# Autodesk Inventor assembly: 000 ASY GBK Gubkinskiy
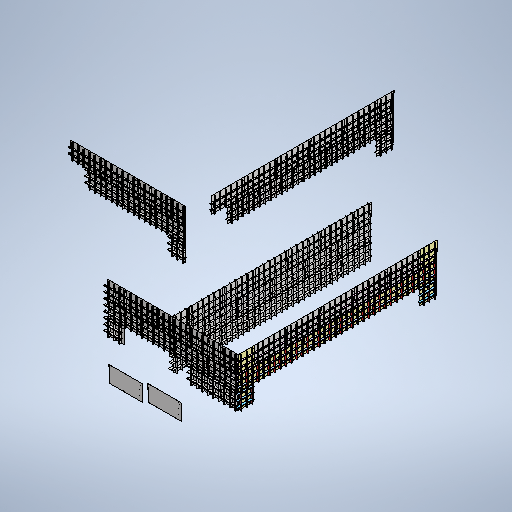
[picture p0: Inventor's stored thumbnail of the model, 512x512]
Saved by Autodesk Inventor 2026.2 (Build 302298010, 298A)
## iProperties
Created: 2026-04-17
Part Number: 000 ASY GBK Gubkinskiy
Document SubType Name: Assembly
Designer: admin
Mass: 2.0116e+07 g
Surface Area: 1.3016e+07 cm^2
Volume: 2.56254e+06 cm^3
Density: 7.85 g/cm^3
Author: admin
## Documents named in this file (20)
- C:\Users\admin\Documents\Inventor\GBK-Gubkinskiy\000 ASY GBK Gubkinskiy.iam
- C:\Users\admin\Documents\Inventor\GBK-Gubkinskiy\GBK bottom.ipt
- C:\Users\admin\Documents\Inventor\GBK-Gubkinskiy\ASY GBK длинная стенка.iam
- C:\Users\admin\Documents\Inventor\GBK-Gubkinskiy\090 ASY bottom.iam
- C:\Users\admin\Documents\Inventor\GBK-Gubkinskiy\ASY GBK короткая стенка.iam
- C:\Users\admin\Documents\Inventor\GBK-Gubkinskiy\ASY GBK центральная стенка.iam
- C:\Users\admin\Documents\Inventor\GBK-Gubkinskiy\ASY GBK 2110 short wall shield 1.iam
- C:\Users\admin\Documents\Inventor\GBK-Gubkinskiy\ASY GBK 2120 short wall shield 2.iam
- C:\Users\admin\Documents\Inventor\GBK-Gubkinskiy\ASY GBK 2130 short wall shield 3.iam
- C:\Users\admin\Documents\Inventor\GBK-Gubkinskiy\ASY GBK 2210 short wall shield 4.iam
- C:\Users\admin\Documents\Inventor\GBK-Gubkinskiy\ASY GBK 2310 short wall shield 7.iam
- C:\Users\admin\Documents\Inventor\GBK-Gubkinskiy\ASY GBK 2320 short wall shield 8.iam
- C:\Users\admin\Documents\Inventor\GBK-Gubkinskiy\ASY GBK 2330 short wall shield 9.iam
- C:\Users\admin\Documents\Inventor\GBK-Gubkinskiy\ASY GBK 2220 short wall shield 5.iam
- C:\Users\admin\Documents\Inventor\GBK-Gubkinskiy\ASY GBK 2230 short wall shield 6.iam
- C:\Users\admin\Documents\Inventor\GBK-Gubkinskiy\ASY GBK 1110 long wall shield 1.iam
- C:\Users\admin\Documents\Inventor\GBK-Gubkinskiy\ASY GBK 1210 long wall shield 3.iam
- C:\Users\admin\Documents\Inventor\GBK-Gubkinskiy\ASY GBK 1310 long wall shield 4.iam
- C:\Users\admin\Documents\Inventor\GBK-Gubkinskiy\ASY GBK 1320 long wall shield 5.iam
- C:\Users\admin\Documents\Inventor\GBK-Gubkinskiy\GBK 2121 shield 2.ipt
## Components (56 placed, 28 different names)
1. GBK bottom.ipt:1 — Flush:8, Flush:9, Mate:20, Mate:21, Flush:14, Mate:23, Flush:19, Flush:21, Flush:22, Mate:24, Mate:25
2. ASY GBK 1110 long wall shield 1.iam:2 [sub-assembly]
3. ASY GBK 1110 long wall shield 1.iam:1 [sub-assembly]
4. ASY GBK 1210 long wall shield 3.iam:1 [sub-assembly]
5. ASY GBK 1310 long wall shield 4.iam:1 [sub-assembly]
6. ASY GBK 1320 long wall shield 5.iam:1 [sub-assembly]
7. ASY GBK 1320 long wall shield 5.iam:2 [sub-assembly]
8. ASY GBK 1320 long wall shield 5.iam:3 [sub-assembly]
9. ASY GBK 1320 long wall shield 5.iam:4 [sub-assembly]
10. ASY GBK 1320 long wall shield 5.iam:5 [sub-assembly]
11. ASY GBK 1210 long wall shield 3.iam:2 [sub-assembly]
12. ASY GBK 1210 long wall shield 3.iam:3 [sub-assembly]
13. ASY GBK 1210 long wall shield 3.iam:4 [sub-assembly]
14. ASY GBK 1210 long wall shield 3.iam:5 [sub-assembly]
15. ASY GBK 1210 long wall shield 3.iam:6 [sub-assembly]
16. ASY GBK 1310 long wall shield 4.iam:2 [sub-assembly]
17. ASY GBK длинная стенка.iam:1 [sub-assembly]
18. ASY GBK длинная стенка.iam:2 [sub-assembly] — Flush:9, Mate:21, Flush:14
19. 090 ASY bottom.iam:1 [sub-assembly] — Mate:19, Flush:8
20. ASY GBK 2110 short wall shield 1.iam:1 [sub-assembly]
21. ASY GBK 2120 short wall shield 2.iam:1 [sub-assembly]
22. ASY GBK 2130 short wall shield 3.iam:1 [sub-assembly]
23. ASY GBK 2210 short wall shield 4.iam:1 [sub-assembly]
24. ASY GBK 2220 short wall shield 5.iam:1 [sub-assembly]
25. ASY GBK 2220 short wall shield 5.iam:2 [sub-assembly]
26. ASY GBK 2230 short wall shield 6.iam:1 [sub-assembly]
27. ASY GBK 2310 short wall shield 7.iam:1 [sub-assembly]
28. ASY GBK 2320 short wall shield 8.iam:1 [sub-assembly]
29. ASY GBK 2330 short wall shield 9.iam:1 [sub-assembly]
30. ASY GBK 2320 short wall shield 8.iam:2 [sub-assembly]
31. ASY GBK 2320 short wall shield 8.iam:3 [sub-assembly]
32. ASY GBK короткая стенка.iam:1 [sub-assembly] — Mate:20, Flush:19, Mate:25, Mate:27
33. ASY GBK короткая стенка.iam:2 [sub-assembly]
34. ASY GBK центральная стенка.iam:1 [sub-assembly] — Mate:23, Flush:18, Mate:27
35. ASY GBK 2110 short wall shield 1:2 [sub-assembly]
36. ASY GBK 2210 short wall shield 4:2 [sub-assembly]
37. ASY GBK 2310 short wall shield 5:2 [sub-assembly]
38. ASY GBK 2320 short wall shield 6:4 [sub-assembly]
39. ASY GBK 2220 short wall shield 5:3 [sub-assembly]
40. ASY GBK 2220 short wall shield 5:4 [sub-assembly]
41. ASY GBK 2320 short wall shield 6:5 [sub-assembly]
42. ASY GBK 2320 short wall shield 6:6 [sub-assembly]
43. ASY GBK 1110 long wall shield 1:3 [sub-assembly]
44. 04 ASY GBK wall shield 1.2.4:7 [sub-assembly]
45. 07 ASY GBK wall shield 1.3.1:3 [sub-assembly]
46. 08 ASY GBK wall shield 1.3.8:6 [sub-assembly]
47. 08 ASY GBK wall shield 1.3.8:7 [sub-assembly]
48. 08 ASY GBK wall shield 1.3.8:8 [sub-assembly]
49. 08 ASY GBK wall shield 1.3.8:9 [sub-assembly]
50. 08 ASY GBK wall shield 1.3.8:10 [sub-assembly]
51. 04 ASY GBK wall shield 1.2.4:8 [sub-assembly]
52. 04 ASY GBK wall shield 1.2.4:9 [sub-assembly]
53. 04 ASY GBK wall shield 1.2.4:10 [sub-assembly]
54. 04 ASY GBK wall shield 1.2.4:11 [sub-assembly]
55. GBK 2121 shield 2:1
56. GBK 2121 shield 2:2
## Relationships (77: WeldJoint 33, Mate 25, Flush 19)
- [Mate]: GBK bottom.ipt:1 ↔ ASY GBK 1110 long wall shield 1.iam:1
- Mate:19: 090 ASY bottom.iam:1
- Flush:8: GBK bottom.ipt:1 ↔ 090 ASY bottom.iam:1
- Flush:9 (-120 mm): GBK bottom.ipt:1 ↔ ASY GBK длинная стенка.iam:2
- Mate:20: GBK bottom.ipt:1 ↔ ASY GBK короткая стенка.iam:1
- Mate:21: GBK bottom.ipt:1 ↔ ASY GBK длинная стенка.iam:2
- Flush:14 (40 mm): GBK bottom.ipt:1 ↔ ASY GBK длинная стенка.iam:2
- [Flush] (40 mm): GBK bottom.ipt:1 ↔ ASY GBK 1110 long wall shield 1.iam:1
- [Mate]: GBK bottom.ipt:1 ↔ ASY GBK 2110 short wall shield 1.iam:1
- [Flush] (40 mm): GBK bottom.ipt:1 ↔ ASY GBK 2110 short wall shield 1.iam:1
- Mate:23: GBK bottom.ipt:1 ↔ ASY GBK центральная стенка.iam:1
- Flush:18 (-2 mm): ASY GBK центральная стенка.iam:1
- Flush:19 (40 mm): GBK bottom.ipt:1 ↔ ASY GBK короткая стенка.iam:1
- [Flush] (120 mm): GBK bottom.ipt:1 ↔ ASY GBK 1110 long wall shield 1.iam:1
- Flush:21: GBK bottom.ipt:1
- Flush:22: GBK bottom.ipt:1
- Mate:24: GBK bottom.ipt:1
- Mate:25 (-360 mm): GBK bottom.ipt:1 ↔ ASY GBK короткая стенка.iam:1
- [Mate] (-360 mm): GBK bottom.ipt:1 ↔ ASY GBK 2130 short wall shield 3.iam:1
- Mate:27 (1.254 mm): ASY GBK короткая стенка.iam:1 ↔ ASY GBK центральная стенка.iam:1
- [WeldJoint] (1 mm): ASY GBK 2110 short wall shield 1.iam:1 ↔ ASY GBK 2120 short wall shield 2.iam:1
- [WeldJoint] (1 mm): ASY GBK 2220 short wall shield 5.iam:1 ↔ ASY GBK 2220 short wall shield 5.iam:2
- [WeldJoint] (1 mm): ASY GBK 2310 short wall shield 7.iam:1 ↔ ASY GBK 2320 short wall shield 8.iam:1
- [WeldJoint] (1 mm): ASY GBK 2320 short wall shield 8.iam:1 ↔ ASY GBK 2320 short wall shield 8.iam:2
- [WeldJoint] (1 mm): ASY GBK 2320 short wall shield 8.iam:2 ↔ ASY GBK 2320 short wall shield 8.iam:3
- [Flush]: ASY GBK 2110 short wall shield 1.iam:1 ↔ ASY GBK короткая стенка.iam:2
- [Flush]: ASY GBK 2110 short wall shield 1.iam:1 ↔ ASY GBK короткая стенка.iam:2
- [Mate]: ASY GBK 2110 short wall shield 1.iam:1 ↔ ASY GBK короткая стенка.iam:2
- [Flush]: ASY GBK 2130 short wall shield 3.iam:1 ↔ ASY GBK 2230 short wall shield 6.iam:1
- [Mate] (1 mm): ASY GBK 2130 short wall shield 3.iam:1 ↔ ASY GBK 2230 short wall shield 6.iam:1
- [Flush]: ASY GBK 2230 short wall shield 6.iam:1 ↔ ASY GBK 2330 short wall shield 9.iam:1
- [Mate] (1 mm): ASY GBK 2230 short wall shield 6.iam:1 ↔ ASY GBK 2330 short wall shield 9.iam:1
- [Mate] (1 mm): ASY GBK 2130 short wall shield 3.iam:1 ↔ ASY GBK 2230 short wall shield 6.iam:1
- [Mate] (1 mm): ASY GBK 2230 short wall shield 6.iam:1 ↔ ASY GBK 2330 short wall shield 9.iam:1
- [WeldJoint] (1 mm): ASY GBK 2330 short wall shield 9.iam:1 ↔ ASY GBK 2320 short wall shield 8.iam:3
- [WeldJoint] (1 mm): ASY GBK 2220 short wall shield 5.iam:2 ↔ ASY GBK 2230 short wall shield 6.iam:1
- [WeldJoint] (1 mm): ASY GBK 2210 short wall shield 4.iam:1 ↔ ASY GBK 2220 short wall shield 5.iam:1
- [WeldJoint] (1 mm): ASY GBK 1210 long wall shield 3.iam:1 ↔ ASY GBK 1210 long wall shield 3.iam:2
- [WeldJoint] (1 mm): ASY GBK 1210 long wall shield 3.iam:2 ↔ ASY GBK 1210 long wall shield 3.iam:3
- [WeldJoint] (1 mm): ASY GBK 1210 long wall shield 3.iam:3 ↔ ASY GBK 1210 long wall shield 3.iam:4
- [WeldJoint] (1 mm): ASY GBK 1210 long wall shield 3.iam:4 ↔ ASY GBK 1210 long wall shield 3.iam:5
- [WeldJoint] (1 mm): ASY GBK 1210 long wall shield 3.iam:5 ↔ ASY GBK 1210 long wall shield 3.iam:6
- [Flush]: ASY GBK 1110 long wall shield 1.iam:1 ↔ ASY GBK длинная стенка.iam:1
- [Mate]: ASY GBK 1110 long wall shield 1.iam:1 ↔ ASY GBK длинная стенка.iam:1
- [Mate]: ASY GBK 1110 long wall shield 1.iam:1 ↔ ASY GBK длинная стенка.iam:1
- [WeldJoint] (1 mm): ASY GBK 1310 long wall shield 4.iam:1 ↔ ASY GBK 1320 long wall shield 5.iam:1
- [WeldJoint] (1 mm): ASY GBK 1320 long wall shield 5.iam:1 ↔ ASY GBK 1320 long wall shield 5.iam:2
- [WeldJoint] (1 mm): ASY GBK 1320 long wall shield 5.iam:2 ↔ ASY GBK 1320 long wall shield 5.iam:3
- [WeldJoint] (1 mm): ASY GBK 1320 long wall shield 5.iam:3 ↔ ASY GBK 1320 long wall shield 5.iam:4
- [WeldJoint] (1 mm): ASY GBK 1320 long wall shield 5.iam:4 ↔ ASY GBK 1320 long wall shield 5.iam:5
- [WeldJoint] (1 mm): ASY GBK 1320 long wall shield 5.iam:5 ↔ ASY GBK 1310 long wall shield 4.iam:2
- [Flush]: ASY GBK 1110 long wall shield 1.iam:1 ↔ ASY GBK 1210 long wall shield 3.iam:1
- [Flush]: ASY GBK 1210 long wall shield 3.iam:1 ↔ ASY GBK 1310 long wall shield 4.iam:1
- [Mate] (1 mm): ASY GBK 1110 long wall shield 1.iam:1 ↔ ASY GBK 1210 long wall shield 3.iam:1
- [Mate] (1 mm): ASY GBK 1210 long wall shield 3.iam:1 ↔ ASY GBK 1310 long wall shield 4.iam:1
- [Mate] (1 mm): ASY GBK 1110 long wall shield 1.iam:1 ↔ ASY GBK 1210 long wall shield 3.iam:1
- [Mate] (1 mm): ASY GBK 1210 long wall shield 3.iam:1 ↔ ASY GBK 1310 long wall shield 4.iam:1
- [WeldJoint] (1 mm): ASY GBK 2220 short wall shield 5:3 ↔ ASY GBK 2220 short wall shield 5:4
- [WeldJoint] (1 mm): ASY GBK 2310 short wall shield 5:2 ↔ ASY GBK 2320 short wall shield 6:4
- [WeldJoint] (1 mm): ASY GBK 2320 short wall shield 6:4 ↔ ASY GBK 2320 short wall shield 6:5
- [WeldJoint] (1 mm): ASY GBK 2320 short wall shield 6:5 ↔ ASY GBK 2320 short wall shield 6:6
- [WeldJoint] (1 mm): ASY GBK 2210 short wall shield 4:2 ↔ ASY GBK 2220 short wall shield 5:3
- [WeldJoint] (1 mm): 04 ASY GBK wall shield 1.2.4:7 ↔ 04 ASY GBK wall shield 1.2.4:8
- [WeldJoint] (1 mm): 04 ASY GBK wall shield 1.2.4:8 ↔ 04 ASY GBK wall shield 1.2.4:9
- [WeldJoint] (1 mm): 04 ASY GBK wall shield 1.2.4:9 ↔ 04 ASY GBK wall shield 1.2.4:10
- [WeldJoint] (1 mm): 04 ASY GBK wall shield 1.2.4:10 ↔ 04 ASY GBK wall shield 1.2.4:11
- [WeldJoint] (1 mm): 07 ASY GBK wall shield 1.3.1:3 ↔ 08 ASY GBK wall shield 1.3.8:6
- [WeldJoint] (1 mm): 08 ASY GBK wall shield 1.3.8:6 ↔ 08 ASY GBK wall shield 1.3.8:7
- [WeldJoint] (1 mm): 08 ASY GBK wall shield 1.3.8:7 ↔ 08 ASY GBK wall shield 1.3.8:8
- [WeldJoint] (1 mm): 08 ASY GBK wall shield 1.3.8:8 ↔ 08 ASY GBK wall shield 1.3.8:9
- [WeldJoint] (1 mm): 08 ASY GBK wall shield 1.3.8:9 ↔ 08 ASY GBK wall shield 1.3.8:10
- [Flush]: ASY GBK 1110 long wall shield 1:3 ↔ 04 ASY GBK wall shield 1.2.4:7
- [Flush]: 04 ASY GBK wall shield 1.2.4:7 ↔ 07 ASY GBK wall shield 1.3.1:3
- [Mate] (1 mm): ASY GBK 1110 long wall shield 1:3 ↔ 04 ASY GBK wall shield 1.2.4:7
- [Mate] (1 mm): 04 ASY GBK wall shield 1.2.4:7 ↔ 07 ASY GBK wall shield 1.3.1:3
- [Mate] (1 mm): ASY GBK 1110 long wall shield 1:3 ↔ 04 ASY GBK wall shield 1.2.4:7
- [Mate] (1 mm): 04 ASY GBK wall shield 1.2.4:7 ↔ 07 ASY GBK wall shield 1.3.1:3
## Named parameters: Зазор_по_горизонту = 1 mm, d120_Зазор_по_горизонту = 1 mm, d141_Зазор_по_горизонту = 1 mm, d159_d141_Зазор_по_горизонту = 1 mm, d175_d141_Зазор_по_горизонту = 1 mm, d249_d19 = 0 mm, d254_Зазор_по_горизонту = 1 mm, d260_d30 = 1 mm, d272_d20 = 0 mm, d274_d22 = 0 mm, d287_d30 = 1 mm, d288_d6 = 1 mm, d289_d9 = 1 mm, d290_d10 = 1 mm, d291_d11 = 1 mm, d298_d254_Зазор_по_горизонту = 1 mm, d304_d260_d30 = 1 mm, d305_d31 = 1 mm, d306_d32 = 1 mm, d307_d33 = 1 mm, d308_d34 = 1 mm, d310_d39 = 0 mm, d311_d40 = 0 mm, d312_d41 = 1 mm, d313_d42 = 1 mm, d314_d43 = 1 mm, d315_d44 = 1 mm
